# Autodesk Inventor assembly: Assembly1
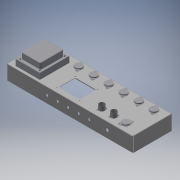
[picture p0: Inventor's stored thumbnail of the model, 180x180]
Saved by Autodesk Inventor 2016 (Build 200138000, 138)
## iProperties
Created: 2015-10-14
Part Number: Assembly1
Document SubType Name: Assembly
Designer: jeremyhale
Author: jeremyhale
## Documents named in this file (5)
- \\psf\Home\Documents\Poorhouse\Amps\p0001\Assembly1.iam
- \\psf\Home\Documents\Poorhouse\Amps\p0001\chassis.ipt
- \\psf\Home\Documents\Poorhouse\Amps\p0001\tube socket 8 pin.ipt
- \\psf\Home\Documents\Poorhouse\Amps\p0001\tube socket 9 pin.ipt
- \\psf\Home\Documents\Poorhouse\Amps\p0001\xmfr power.ipt
## Components (11 placed, 4 different names)
1. chassis:1 — Rotational:1, Rotational:2, Rotational:3, Rotational:4, Rotational:5, Rotational:6, Rotational:7, Rotational:8
2. tube socket 8 pin:7 — Rotational:3, Rotational:4
3. xmfr power:1 — Rotational:7, Rotational:8
4. tube socket 8 pin:1 — Rotational:1, Rotational:2
5. tube socket 8 pin:2
6. tube socket 8 pin:3
7. tube socket 8 pin:4
8. tube socket 8 pin:5
9. tube socket 8 pin:6
10. tube socket 9 pin:1 — Rotational:5, Rotational:6
11. tube socket 9 pin:2
## Component patterns: Big Tube Sockets (6 elements), (2 elements, first: tube socket 9 pin:1)
## Relationships (8: RevoluteJoint 8)
- Rotational:1 [RevoluteJoint]: chassis:1 ↔ tube socket 8 pin:1
- Rotational:2 [RevoluteJoint]: chassis:1 ↔ tube socket 8 pin:1
- Rotational:3 [RevoluteJoint]: chassis:1 ↔ tube socket 8 pin:7
- Rotational:4 [RevoluteJoint]: chassis:1 ↔ tube socket 8 pin:7
- Rotational:5 [RevoluteJoint]: chassis:1 ↔ tube socket 9 pin:1
- Rotational:6 [RevoluteJoint]: chassis:1 ↔ tube socket 9 pin:1
- Rotational:7 [RevoluteJoint]: chassis:1 ↔ xmfr power:1
- Rotational:8 [RevoluteJoint]: chassis:1 ↔ xmfr power:1
